# Autodesk Inventor assembly: ASY SLM 1110 MAIN FRAME
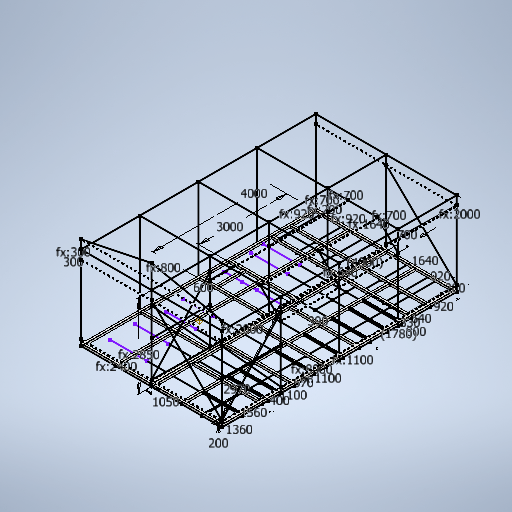
[picture p0: Inventor's stored thumbnail of the model, 512x512]
Saved by Autodesk Inventor 2025 (Build 290162010, 162A)
## iProperties
Created: 2025-12-15
Part Number: ASY SLM 1110 MAIN FRAME
Document SubType Name: Assembly
Designer: admin
Mass: 1.03915e+06 g
Surface Area: 883173 cm^2
Volume: 132376 cm^3
Density: 7.85 g/cm^3
_SolveAssemblyDoc: Frame Generator Solve Assembly
_Version: 25.0.0
Author: admin
## Documents named in this file (15)
- C:\Users\admin\Yandex.Disk\home pc\Inventor\SLM-Salemal\ASY SLM 1110 MAIN FRAME.iam
- C:\Users\admin\Yandex.Disk\home pc\Inventor\SLM-Salemal\Frame\PNS-1100 FRAME Main sketch.ipt
- C:\Users\admin\Yandex.Disk\home pc\Inventor\SLM-Salemal\ASY SLM 1110 MAIN FRAME\Frame\Frame 1768306688236.iam
- C:\Users\admin\Yandex.Disk\home pc\Inventor\SLM-Salemal\SLM-frame 1.1 floor sheet 4.ipt
- C:\Users\admin\Yandex.Disk\home pc\Inventor\SLM-Salemal\SLM-frame 1.1 floor sheet 5.ipt
- C:\Users\admin\Yandex.Disk\home pc\Inventor\SLM-Salemal\SLM-frame 1.1 floor sheet 4_CPY.ipt
- C:\Users\admin\Yandex.Disk\home pc\Inventor\SLM-Salemal\SLM-frame 1.1 floor sheet 2.ipt
- C:\Users\admin\Yandex.Disk\home pc\Inventor\SLM-Salemal\SLM-frame 1.1 floor sheet 3.ipt
- C:\Users\admin\Yandex.Disk\home pc\Inventor\SLM-Salemal\SLM-frame 1.1 floor sheet.ipt
- C:\Users\admin\Yandex.Disk\home pc\Inventor\SLM-Salemal\SLM-frame 2 floor sheet 5.ipt
- C:\Users\admin\Yandex.Disk\home pc\Inventor\SLM-Salemal\SLM-frame 2 floor sheet 6.ipt
- C:\Users\admin\Yandex.Disk\home pc\Inventor\SLM-Salemal\SLM-frame 2 floor sheet 7.ipt
- C:\Users\admin\Yandex.Disk\home pc\Inventor\SLM-Salemal\SLM-frame 2 floor sheet 8.ipt
- C:\Users\admin\Yandex.Disk\home pc\Inventor\SLM-Salemal\SLM-frame 2 floor sheet 9.ipt
- C:\Users\admin\Yandex.Disk\home pc\Inventor\SLM-Salemal\SLM-frame 2 floor sheet 10.ipt
## Components (27 placed, 20 different names)
1. PNS-1100 FRAME Main sketch.ipt:1
2. Frame 1768306688236.iam:1 [sub-assembly] — Mate:1, Mate:2, Mate:3
3. SLM-frame 1.1 floor sheet.ipt:1 — Mate:1, Mate:2, Mate:3, Rigid:3, Rigid:17
4. SLM-frame 1.1 floor sheet 2.ipt:1 — Rigid:3, Rigid:4
5. SLM-frame 1.1 floor sheet 4.ipt:1 — Rigid:1, Rigid:5
6. SLM-frame 1.1 floor sheet 5.ipt:1 — Rigid:1, Rigid:9
7. SLM-frame 1.1 floor sheet 4_CPY.ipt:1
8. SLM-frame 1.1 floor sheet 3.ipt:1 — Rigid:4, Rigid:5
9. SLM-frame 1.1 floor sheet 4.ipt:2
10. SLM-frame 1.1 floor sheet 4_CPY.ipt:2
11. SLM-frame 1.1 floor sheet 5.ipt:2
12. SLM-frame 2 floor sheet 5.ipt:1
13. SLM-frame 2 floor sheet 6.ipt:1
14. SLM-frame 2 floor sheet 7.ipt:1
15. SLM-frame 2 floor sheet 8.ipt:1
16. SLM-frame 2 floor sheet 9.ipt:1
17. SLM-frame 2 floor sheet 10.ipt:1 — Rigid:6, Rigid:9
18. SLM-frame 2 floor sheet 10:2 — Rigid:6, Rigid:7
19. SLM-frame 2 floor sheet 10:3 — Rigid:7
20. SLM-frame 1.1 floor sheet 4:3
21. SLM-frame 1.1 floor sheet 5:3
22. SLM-frame 1.1 floor sheet 2:2
23. SLM-frame 1.1 floor sheet 3:2
24. Part1:3 — Rigid:17
25. SLM-frame 2 floor sheet 10:4
26. SLM-frame 2 floor sheet 10:5
27. SLM-frame 2 floor sheet 10:6
## Relationships (18: WeldJoint 15, Mate 3)
- Rigid:1 [WeldJoint] (20 mm): SLM-frame 1.1 floor sheet 4.ipt:1 ↔ SLM-frame 1.1 floor sheet 5.ipt:1
- Mate:1: Frame 1768306688236.iam:1 ↔ SLM-frame 1.1 floor sheet.ipt:1
- Mate:2 (-30 mm): Frame 1768306688236.iam:1 ↔ SLM-frame 1.1 floor sheet.ipt:1
- Mate:3 (-30 mm): Frame 1768306688236.iam:1 ↔ SLM-frame 1.1 floor sheet.ipt:1
- Rigid:3 [WeldJoint] (20 mm): SLM-frame 1.1 floor sheet.ipt:1 ↔ SLM-frame 1.1 floor sheet 2.ipt:1
- Rigid:4 [WeldJoint] (20 mm): SLM-frame 1.1 floor sheet 2.ipt:1 ↔ SLM-frame 1.1 floor sheet 3.ipt:1
- Rigid:5 [WeldJoint] (20 mm): SLM-frame 1.1 floor sheet 4.ipt:1 ↔ SLM-frame 1.1 floor sheet 3.ipt:1
- Rigid:6 [WeldJoint] (20 mm): SLM-frame 2 floor sheet 10.ipt:1 ↔ SLM-frame 2 floor sheet 10:2
- Rigid:7 [WeldJoint] (20 mm): SLM-frame 2 floor sheet 10:2 ↔ SLM-frame 2 floor sheet 10:3
- Rigid:9 [WeldJoint] (20 mm): SLM-frame 1.1 floor sheet 5.ipt:1 ↔ SLM-frame 2 floor sheet 10.ipt:1
- [WeldJoint] (20 mm): SLM-frame 1.1 floor sheet 4:3 ↔ SLM-frame 1.1 floor sheet 5:3
- [WeldJoint] (20 mm): SLM-frame 1.1 floor sheet 2:2 ↔ Part1:3
- [WeldJoint] (20 mm): SLM-frame 1.1 floor sheet 2:2 ↔ SLM-frame 1.1 floor sheet 3:2
- [WeldJoint] (20 mm): SLM-frame 1.1 floor sheet 4:3 ↔ SLM-frame 1.1 floor sheet 3:2
- [WeldJoint] (20 mm): SLM-frame 2 floor sheet 10:4 ↔ SLM-frame 2 floor sheet 10:5
- [WeldJoint] (20 mm): SLM-frame 2 floor sheet 10:5 ↔ SLM-frame 2 floor sheet 10:6
- [WeldJoint] (20 mm): SLM-frame 1.1 floor sheet 5:3 ↔ SLM-frame 2 floor sheet 10:4
- Rigid:17 [WeldJoint] (100 mm): SLM-frame 1.1 floor sheet.ipt:1 ↔ Part1:3
